# Autodesk Inventor assembly: DynamixelXM540_drivable
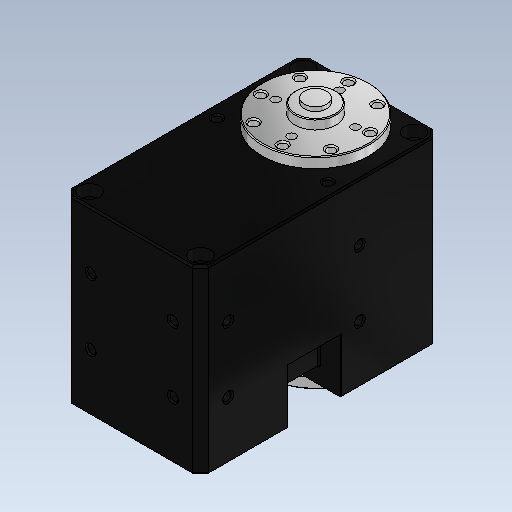
[picture p0: Inventor's stored thumbnail of the model, 512x512]
Saved by Autodesk Inventor 2023 (Build 270158000, 158)
## iProperties
Created: 2018-06-30
Part Number: DynamixelXM540_drivable
Material: 一般
Document SubType Name: Assembly
Designer: TAKEMORI
Mass: 160.724 g
Surface Area: 218.4 cm^2
Volume: 59.5273 cm^3
Density: 2.7 g/cm^3
Author: TAKEMORI
## Documents named in this file (4)
- C:\Users\michi\OneDrive - Kyoto University\lab\6_SHINOBI\FUHGA4\Design_Mechanism\00_devices\Dynamixel\X540\DynamixelXM540_drivable.iam
- C:\Users\michi\OneDrive - Kyoto University\lab\6_SHINOBI\FUHGA3\Design_Mechanism\Dynamixel\X540\DynamixelXM540_without_hone.ipt
- C:\Users\michi\OneDrive - Kyoto University\lab\6_SHINOBI\FUHGA3\Design_Mechanism\Dynamixel\X540\DynamixelXM540_hone.ipt
- C:\Users\michi\OneDrive - Kyoto University\lab\6_SHINOBI\FUHGA3\Design_Mechanism\Dynamixel\X540\DynamixelXM540_idler.ipt
## Components (3 placed, 3 different names)
1. DynamixelXM540_without_hone:1 — フラッシュ:1, フラッシュ:2, フラッシュ:3, 挿入:1, 挿入:2
2. DynamixelXM540_hone:1 — 挿入:1
3. DynamixelXM540_idler:1 — 挿入:2
## Relationships (5: Flush 3, Insert 2)
- フラッシュ:1 [Flush]: DynamixelXM540_without_hone:1
- フラッシュ:2 [Flush]: DynamixelXM540_without_hone:1
- フラッシュ:3 [Flush]: DynamixelXM540_without_hone:1
- 挿入:1 [Insert]: DynamixelXM540_without_hone:1 ↔ DynamixelXM540_hone:1
- 挿入:2 [Insert]: DynamixelXM540_without_hone:1 ↔ DynamixelXM540_idler:1
